# Autodesk Inventor assembly: Differential Swerve Drive V2
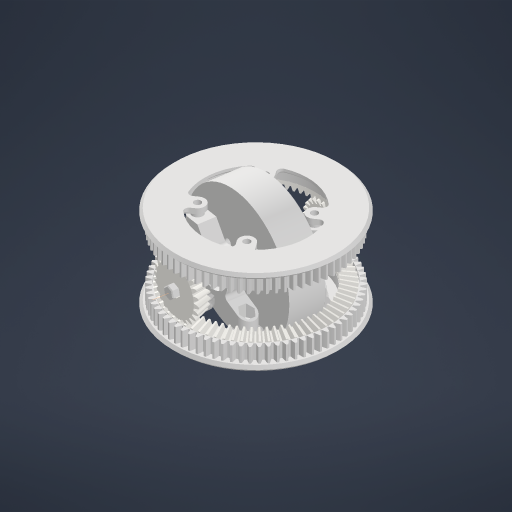
[picture p0: Inventor's stored thumbnail of the model, 512x512]
Saved by Autodesk Inventor 2024 (Build 280153000, 153)
## iProperties
Created: 2023-08-25
Part Number: Differential Swerve Drive V2
Document SubType Name: Assembly
Designer: Izack Waczko
Author: Izack Waczko
## Documents named in this file (8)
- C:\Users\izack\Robotics\CAD\Custom-Modules-CAD\Differential Swerve Drive V1\Differential Swerve Drive V2.iam
- C:\Users\izack\Robotics\CAD\Custom-Modules-CAD\Differential Swerve Drive V1\Differential Swerve Drive Parts\Ring Gear.iam
- C:\Users\izack\Robotics\CAD\Custom-Modules-CAD\Differential Swerve Drive V1\Differential Swerve Drive Parts\Top_Ring_Gear.iam
- C:\Users\izack\Robotics\CAD\Custom-Modules-CAD\Differential Swerve Drive V1\Differential Swerve Drive Parts\Center_Bracket.ipt
- C:\Users\izack\Robotics\CAD\Custom-Modules-CAD\Differential Swerve Drive V1\Differential Swerve Drive Parts\V-Groove Bearing.ipt
- C:\Users\izack\Robotics\CAD\Custom-Modules-CAD\Differential Swerve Drive V1\Differential Swerve Drive Parts\60mm_ThinWheel.ipt
- C:\Users\izack\Robotics\CAD\Custom-Modules-CAD\Differential Swerve Drive V1\Differential Swerve Drive Parts\5mm x 55mm Hex Shaft.ipt
- C:\Users\izack\Robotics\CAD\Custom-Modules-CAD\Differential Swerve Drive V1\Differential Swerve Drive V1\Design Accelerator\Bevel Gear21.ipt
## Components (12 placed, 7 different names)
1. Ring Gear:1 [sub-assembly] — Mate:1, Mate:4, Mate:5
2. Top_Ring_Gear:1 [sub-assembly] — Mate:4, Mate:5, Mate:6, Rigid:1, Rigid:3
3. Center_Bracket:1 — Mate:6, Rigid:1, Rotational:3, Rotational:4
4. Center_Bracket:2 — Rigid:3, Rotational:2, Rigid:2, Mate:7, Mate:8
5. V-Groove Bearing:1 — Rotational:2
6. V-Groove Bearing:2 — Rigid:2
7. V-Groove Bearing:3 — Rotational:3
8. V-Groove Bearing:4 — Rotational:4
9. 60mm_ThinWheel:1 — Mate:7, Mate:8, Mate:9, Mate:10
10. 5mm x 55mm Hex Shaft:1 — Mate:9, Mate:10, Mate:11, Mate:12, Mate:13, Mate:14
11. Bevel Gear2:1 — Mate:11, Mate:12
12. Bevel Gear2:2 — Mate:13, Mate:14
## Relationships (18: Mate 12, WeldJoint 3, RevoluteJoint 3)
- Mate:1: Ring Gear:1
- Mate:4 (-41 mm): Ring Gear:1 ↔ Top_Ring_Gear:1
- Mate:5: Ring Gear:1 ↔ Top_Ring_Gear:1
- Mate:6: Top_Ring_Gear:1 ↔ Center_Bracket:1
- Rigid:1 [WeldJoint]: Top_Ring_Gear:1 ↔ Center_Bracket:1
- Rigid:3 [WeldJoint]: Top_Ring_Gear:1 ↔ Center_Bracket:2
- Rotational:2 [RevoluteJoint]: Center_Bracket:2 ↔ V-Groove Bearing:1
- Rigid:2 [WeldJoint]: Center_Bracket:2 ↔ V-Groove Bearing:2
- Rotational:3 [RevoluteJoint]: Center_Bracket:1 ↔ V-Groove Bearing:3
- Rotational:4 [RevoluteJoint]: Center_Bracket:1 ↔ V-Groove Bearing:4
- Mate:7: Center_Bracket:2 ↔ 60mm_ThinWheel:1
- Mate:8 (2.5 mm): Center_Bracket:2 ↔ 60mm_ThinWheel:1
- Mate:9: 60mm_ThinWheel:1 ↔ 5mm x 55mm Hex Shaft:1
- Mate:10: 60mm_ThinWheel:1 ↔ 5mm x 55mm Hex Shaft:1
- Mate:11: 5mm x 55mm Hex Shaft:1 ↔ Bevel Gear2:1
- Mate:12: 5mm x 55mm Hex Shaft:1 ↔ Bevel Gear2:1
- Mate:13: 5mm x 55mm Hex Shaft:1 ↔ Bevel Gear2:2
- Mate:14: 5mm x 55mm Hex Shaft:1 ↔ Bevel Gear2:2
